# Autodesk Inventor assembly: Diff_test
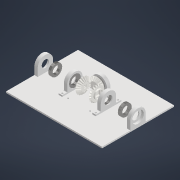
[picture p0: Inventor's stored thumbnail of the model, 180x180]
Saved by Autodesk Inventor 2021 (Build 250183000, 183)
## iProperties
Created: 2021-01-24
Part Number: Diff_test
Document SubType Name: Assembly
Designer: Ctroi
Author: Ctroi
## Documents named in this file (5)
- G:\Roverprojekt\Github Projekt\Rover\Diff_test.iam
- G:\Roverprojekt\Github Projekt\Rover\Testplatte_Differential.ipt
- G:\Roverprojekt\Github Projekt\Rover\Halterung_Differential.ipt
- G:\Roverprojekt\Github Projekt\Rover\Kegelrad.ipt
- G:\Roverprojekt\Github Projekt\Rover\Kugellager.ipt
## Components (12 placed, 4 different names)
1. Testplatte_Differential:1 — Passend:1, Passend:2, Passend:3, Passend:4, Passend:5, Passend:6, Passend:7, Passend:8, Passend:13, Passend:14, Passend:15, Passend:16, Passend:17
2. Halterung_Differential:1 — Passend:1, Passend:2, Passend:3, Passend:11, Passend:12
3. Halterung_Differential:2 — Passend:4, Passend:5, Passend:6, Passend:9, Passend:10
4. Kegelrad2:1
5. Kegelrad2:2
6. Kegelrad2:3
7. Kugellager:1 — Passend:7, Passend:8
8. Kugellager:2 — Passend:9, Passend:10
9. Kugellager:3 — Passend:11, Passend:12
10. Kugellager:4 — Passend:13, Passend:14
11. Halterung_Differential:3 — Passend:15, Passend:16, Passend:17, Passend:18, Passend:19
12. Kugellager:5 — Passend:18, Passend:19
## Relationships (19: Mate 19)
- Passend:1 [Mate]: Testplatte_Differential:1 ↔ Halterung_Differential:1
- Passend:2 [Mate]: Testplatte_Differential:1 ↔ Halterung_Differential:1
- Passend:3 [Mate]: Testplatte_Differential:1 ↔ Halterung_Differential:1
- Passend:4 [Mate]: Testplatte_Differential:1 ↔ Halterung_Differential:2
- Passend:5 [Mate]: Testplatte_Differential:1 ↔ Halterung_Differential:2
- Passend:6 [Mate]: Testplatte_Differential:1 ↔ Halterung_Differential:2
- Passend:7 [Mate]: Testplatte_Differential:1 ↔ Kugellager:1
- Passend:8 [Mate]: Testplatte_Differential:1 ↔ Kugellager:1
- Passend:9 [Mate]: Halterung_Differential:2 ↔ Kugellager:2
- Passend:10 [Mate]: Halterung_Differential:2 ↔ Kugellager:2
- Passend:11 [Mate]: Halterung_Differential:1 ↔ Kugellager:3
- Passend:12 [Mate]: Halterung_Differential:1 ↔ Kugellager:3
- Passend:13 [Mate]: Testplatte_Differential:1 ↔ Kugellager:4
- Passend:14 [Mate]: Testplatte_Differential:1 ↔ Kugellager:4
- Passend:15 [Mate]: Testplatte_Differential:1 ↔ Halterung_Differential:3
- Passend:16 [Mate]: Testplatte_Differential:1 ↔ Halterung_Differential:3
- Passend:17 [Mate]: Testplatte_Differential:1 ↔ Halterung_Differential:3
- Passend:18 [Mate]: Halterung_Differential:3 ↔ Kugellager:5
- Passend:19 [Mate]: Halterung_Differential:3 ↔ Kugellager:5
